# Autodesk Inventor assembly: flute
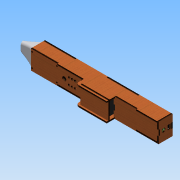
[picture p0: Inventor's stored thumbnail of the model, 180x180]
Saved by Autodesk Inventor 2015 (Build 190159000, 159)
## iProperties
Created: 2015-12-28
Part Number: flute
Document SubType Name: Assembly
Designer: Gregwar
Author: Gregwar
## Documents named in this file (10)
- C:\Users\Gregwar\Desktop\eFlute\3d\v1\flute.iam
- C:\Users\Gregwar\Desktop\eFlute\3d\v1\electronics.ipt
- C:\Users\Gregwar\Desktop\eFlute\3d\v1\bec.ipt
- C:\Users\Gregwar\Desktop\eFlute\3d\v1\top.ipt
- C:\Users\Gregwar\Desktop\eFlute\3d\v1\side.ipt
- C:\Users\Gregwar\Desktop\eFlute\3d\v1\bottom.ipt
- C:\Users\Gregwar\Desktop\eFlute\3d\v1\bottom_renfort.ipt
- C:\Users\Gregwar\Desktop\eFlute\3d\v1\connectors.ipt
- C:\Users\Gregwar\Desktop\eFlute\3d\v1\bottom2.ipt
- C:\Users\Gregwar\Desktop\eFlute\3d\v1\cache.ipt
## Components (10 placed, 9 different names)
1. electronics:1 — Placage:1, Placage:2, Placage:3
2. bec:1 — Placage:1, Placage:2, Placage:3, Placage:4, Placage:5, Placage:6, Placage:10, Placage:11
3. top:1 — Placage:4, Placage:5, Placage:6, Placage:7, Affleurement:1, Affleurement:2, Placage:8, Affleurement:3, Affleurement:4, Placage:14, Affleurement:6
4. side:1 — Placage:7, Affleurement:1, Affleurement:2, Affleurement:7, Placage:18
5. side:2 — Placage:8, Affleurement:3, Affleurement:4, Placage:9, Placage:15, Affleurement:9, Placage:16, Affleurement:10, Placage:17
6. bottom:1 — Placage:9, Placage:10, Placage:11, Placage:12, Affleurement:5, Placage:13
7. bottom_renfort:1 — Placage:12, Affleurement:5, Placage:13
8. connectors:1 — Placage:14, Affleurement:6, Affleurement:7, Affleurement:8
9. bottom2:1 — Placage:15, Affleurement:8, Affleurement:9
10. cache:1 — Placage:16, Affleurement:10, Placage:17, Placage:18
## Relationships (28: Mate 18, Flush 10)
- Placage:1 [Mate]: electronics:1 ↔ bec:1
- Placage:2 [Mate]: electronics:1 ↔ bec:1
- Placage:3 [Mate]: electronics:1 ↔ bec:1
- Placage:4 [Mate]: bec:1 ↔ top:1
- Placage:5 [Mate]: bec:1 ↔ top:1
- Placage:6 [Mate]: bec:1 ↔ top:1
- Placage:7 [Mate]: top:1 ↔ side:1
- Affleurement:1 [Flush]: top:1 ↔ side:1
- Affleurement:2 [Flush]: top:1 ↔ side:1
- Placage:8 [Mate]: top:1 ↔ side:2
- Affleurement:3 [Flush]: top:1 ↔ side:2
- Affleurement:4 [Flush]: top:1 ↔ side:2
- Placage:9 [Mate]: side:2 ↔ bottom:1
- Placage:10 [Mate]: bec:1 ↔ bottom:1
- Placage:11 [Mate]: bec:1 ↔ bottom:1
- Placage:12 [Mate]: bottom:1 ↔ bottom_renfort:1
- Affleurement:5 [Flush]: bottom:1 ↔ bottom_renfort:1
- Placage:13 [Mate]: bottom:1 ↔ bottom_renfort:1
- Placage:14 [Mate]: top:1 ↔ connectors:1
- Affleurement:6 [Flush]: top:1 ↔ connectors:1
- Affleurement:7 [Flush]: side:1 ↔ connectors:1
- Placage:15 [Mate]: side:2 ↔ bottom2:1
- Affleurement:8 [Flush]: connectors:1 ↔ bottom2:1
- Affleurement:9 [Flush]: side:2 ↔ bottom2:1
- Placage:16 [Mate]: side:2 ↔ cache:1
- Affleurement:10 [Flush]: side:2 ↔ cache:1
- Placage:17 [Mate]: side:2 ↔ cache:1
- Placage:18 [Mate]: side:1 ↔ cache:1
